# Autodesk Inventor assembly: MolexFixClip_Assy
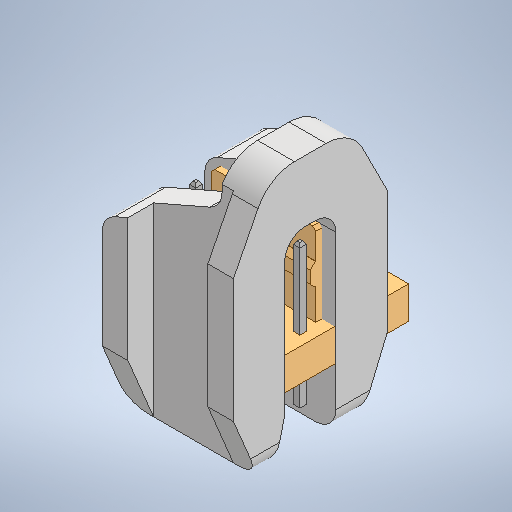
[picture p0: Inventor's stored thumbnail of the model, 512x512]
Saved by Autodesk Inventor 2025.1 (Build 291241000, 241)
## iProperties
Created: 2026-05-09
Part Number: MolexFixClip_Assy
Document SubType Name: Assembly
Designer: User
Author: User
## Documents named in this file (6)
- D:\One Drive\OneDrive - Politeknik Sultan Salahuddin Abdul Aziz Shah\Documents\Inventor\RobosotPSA\MolexFixClip_Assy.iam
- D:\One Drive\OneDrive - Politeknik Sultan Salahuddin Abdul Aziz Shah\Documents\Inventor\RobosotPSA\Molex-2.54-5pin\Molex-2.54-5pin\Molex-2.54-5pin.ipt
- D:\One Drive\OneDrive - Politeknik Sultan Salahuddin Abdul Aziz Shah\Documents\Inventor\RobosotPSA\MolexClipper.ipt
- D:\One Drive\OneDrive - Politeknik Sultan Salahuddin Abdul Aziz Shah\Documents\Inventor\RobosotPSA\MolexClipper_vertical.ipt
- D:\One Drive\OneDrive - Politeknik Sultan Salahuddin Abdul Aziz Shah\Documents\Inventor\RobosotPSA\MolexClipper_v2.ipt
- D:\One Drive\OneDrive - Politeknik Sultan Salahuddin Abdul Aziz Shah\Documents\Inventor\RobosotPSA\MolexClipper_v3.ipt
## Components (6 placed, 5 different names)
1. Molex-2.54-5pin:1 — Flush:1, Flush:2, Flush:3, Flush:4, Mate:1, Mate:2, Flush:5, Mate:3, Flush:6, Mate:4, Mate:5
2. MolexClipper:1 — Flush:1
3. MolexClipper_vertical:1 — Flush:2
4. Molex-2.54-5pin:2 — Flush:3, Flush:4, Mate:1
5. MolexClipper_v2:1 — Mate:2, Flush:5, Mate:3
6. MolexClipper_v3:1 — Flush:6, Mate:4, Mate:5
## Relationships (11: Flush 6, Mate 5)
- Flush:1: Molex-2.54-5pin:1 ↔ MolexClipper:1
- Flush:2: Molex-2.54-5pin:1 ↔ MolexClipper_vertical:1
- Flush:3: Molex-2.54-5pin:1 ↔ Molex-2.54-5pin:2
- Flush:4: Molex-2.54-5pin:1 ↔ Molex-2.54-5pin:2
- Mate:1 (1 mm): Molex-2.54-5pin:1 ↔ Molex-2.54-5pin:2
- Mate:2 (0.1 mm): Molex-2.54-5pin:1 ↔ MolexClipper_v2:1
- Flush:5: Molex-2.54-5pin:1 ↔ MolexClipper_v2:1
- Mate:3 (0.1 mm): Molex-2.54-5pin:1 ↔ MolexClipper_v2:1
- Flush:6: Molex-2.54-5pin:1 ↔ MolexClipper_v3:1
- Mate:4 (0.1 mm): Molex-2.54-5pin:1 ↔ MolexClipper_v3:1
- Mate:5: Molex-2.54-5pin:1 ↔ MolexClipper_v3:1
